# Autodesk Inventor assembly: Y-Idler2
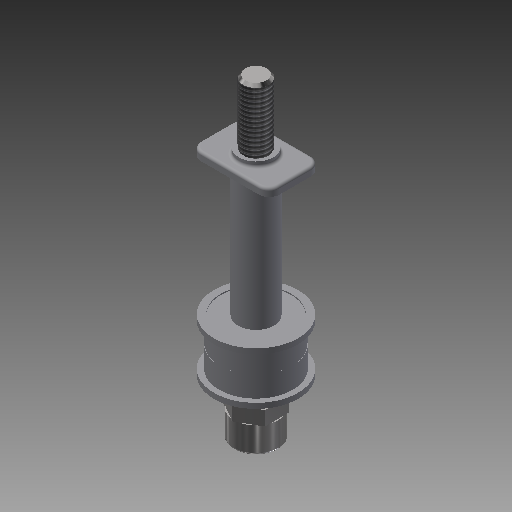
[picture p0: Inventor's stored thumbnail of the model, 512x512]
Saved by Autodesk Inventor 2018 (Build 220112000, 112)
## iProperties
Created: 2016-08-03
Part Number: Y-Idler2
Document SubType Name: Assembly
Designer: User
Author: User
## Documents named in this file (6)
- C:\Users\Dan\OneDrive\SL-Inventor\The Beast v1.2 PackandGo\Workspaces\Workspace\Y-Idler2.iam
- C:\Users\Dan\OneDrive\SL-Inventor\The Beast v1.2 PackandGo\Workspaces\Workspace\M5 Tee Nut-Generic_MIR.ipt
- C:\Users\Dan\OneDrive\SL-Inventor\The Beast v1.2 PackandGo\Workspaces\Workspace\Flanged Bearing_CPY_MIR.ipt
- C:\Users\Dan\OneDrive\SL-Inventor\The Beast v1.2 PackandGo\Workspaces\Workspace\en-US\CSN EN 24 036\CSN EN 24 036 - M5.ipt
- C:\Users\Dan\OneDrive\SL-Inventor\The Beast v1.2 PackandGo\Workspaces\Workspace\25mmspacer_MIR.ipt
- C:\Users\Dan\OneDrive\SL-Inventor\The Beast v1.2 PackandGo\Workspaces\Workspace\en-US\ANSI B18.3.1M(6)\ANSI B18.3.1M - M5x0.8 x 50(1).ipt
## Components (7 placed, 5 different names)
1. Forged Socket Head Cap Screw - Metric M5x0.8 x 50:1 — Mate:10
2. M5 Tee Nut-Generic_MIR:1
3. Flanged Bearing_CPY_MIR:1 — Mate:13
4. Flanged Bearing_CPY_MIR:2 — Mate:14
5. CSN EN 24036 M5:1 — Mate:11
6. 25mmspacer_MIR:1 — Mate:14
7. CSN EN 24036 M5:2 — Mate:10, Mate:11, Mate:13
## Relationships (12: Mate 12)
- [Mate]: Forged Socket Head Cap Screw - Metric M5x0.8 x 50:1 ↔ M5 Tee Nut-Generic_MIR:1
- [Mate]: Forged Socket Head Cap Screw - Metric M5x0.8 x 50:1 ↔ Flanged Bearing_CPY_MIR:1
- [Mate]: Flanged Bearing_CPY_MIR:1 ↔ Flanged Bearing_CPY_MIR:2
- [Mate]: Forged Socket Head Cap Screw - Metric M5x0.8 x 50:1 ↔ Flanged Bearing_CPY_MIR:2
- [Mate]: Forged Socket Head Cap Screw - Metric M5x0.8 x 50:1 ↔ CSN EN 24036 M5:1
- [Mate]: Forged Socket Head Cap Screw - Metric M5x0.8 x 50:1 ↔ CSN EN 24036 M5:1
- [Mate]: Forged Socket Head Cap Screw - Metric M5x0.8 x 50:1 ↔ 25mmspacer_MIR:1
- [Mate]: M5 Tee Nut-Generic_MIR:1 ↔ 25mmspacer_MIR:1
- Mate:10: Forged Socket Head Cap Screw - Metric M5x0.8 x 50:1 ↔ CSN EN 24036 M5:2
- Mate:11: CSN EN 24036 M5:1 ↔ CSN EN 24036 M5:2
- Mate:13: Flanged Bearing_CPY_MIR:1 ↔ CSN EN 24036 M5:2
- Mate:14: Flanged Bearing_CPY_MIR:2 ↔ 25mmspacer_MIR:1
